# Autodesk Inventor assembly: link1
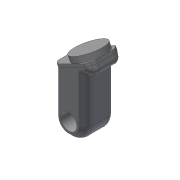
[picture p0: Inventor's stored thumbnail of the model, 180x180]
Saved by Autodesk Inventor 2018 (Build 220112000, 112)
## iProperties
Created: 2019-11-23
Part Number: link1
Document SubType Name: Assembly
Designer: Clevo
Author: Clevo
## Documents named in this file (3)
- E:\RobotArm\Software\URDF_Files\link1.iam
- E:\RobotArm\Software\URDF_Files\arm1.ipt
- E:\RobotArm\Software\URDF_Files\table.ipt
## Components (2 placed, 2 different names)
1. arm1:1 — Flush:1, Flush:2, Mate:1
2. table:1 — Flush:1, Flush:2, Mate:1
## Relationships (3: Flush 2, Mate 1)
- Flush:1: arm1:1 ↔ table:1
- Flush:2: arm1:1 ↔ table:1
- Mate:1: arm1:1 ↔ table:1
